# Autodesk Inventor assembly: GrampoParalelo
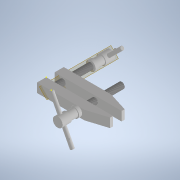
[picture p0: Inventor's stored thumbnail of the model, 180x180]
Saved by Autodesk Inventor 2021 (Build 250183000, 183)
## iProperties
Created: 2022-03-08
Part Number: GrampoParalelo
Document SubType Name: Assembly
Designer: aluno
Author: aluno
## Documents named in this file (6)
- E:\SENAI\Terceiro semestre\TPMC - Tecnololgia de produção mecatrônica\Grampo paralelo\GrampoParalelo.iam
- E:\SENAI\Terceiro semestre\TPMC - Tecnololgia de produção mecatrônica\Grampo paralelo\Garra2.ipt
- E:\SENAI\Terceiro semestre\TPMC - Tecnololgia de produção mecatrônica\Grampo paralelo\Parafuso2.ipt
- E:\SENAI\Terceiro semestre\TPMC - Tecnololgia de produção mecatrônica\Grampo paralelo\Garra1.ipt
- E:\SENAI\Terceiro semestre\TPMC - Tecnololgia de produção mecatrônica\Grampo paralelo\Parafuso1.ipt
- E:\SENAI\Terceiro semestre\TPMC - Tecnololgia de produção mecatrônica\Grampo paralelo\Manipulo.iam
## Components (6 placed, 5 different names)
1. Garra2:1 — Coincidente:1, Coincidente:3
2. Parafuso2:1 — Coincidente:1, Inserir:1, Tangente:1, Coincidente:6, Alinhado:2
3. Garra1:1 — Inserir:1, Coincidente:2, Coincidente:4, Tangente:1
4. Parafuso1:1 — Coincidente:2, Coincidente:3, Coincidente:4, Coincidente:5, Alinhado:1
5. Manipulo:1 [sub-assembly] — Coincidente:6, Alinhado:2
6. Manipulo:2 [sub-assembly] — Coincidente:5, Alinhado:1
## Relationships (10: Mate 6, Flush 2, Insert 1, Tangent 1)
- Coincidente:1 [Mate]: Garra2:1 ↔ Parafuso2:1
- Inserir:1: Parafuso2:1 ↔ Garra1:1
- Coincidente:2 [Mate]: Garra1:1 ↔ Parafuso1:1
- Coincidente:3 [Mate]: Garra2:1 ↔ Parafuso1:1
- Coincidente:4 [Mate]: Garra1:1 ↔ Parafuso1:1
- Tangente:1: Parafuso2:1 ↔ Garra1:1
- Coincidente:5 [Mate]: Parafuso1:1 ↔ Manipulo:2
- Alinhado:1 [Flush] (37.5 mm): Parafuso1:1 ↔ Manipulo:2
- Coincidente:6 [Mate]: Parafuso2:1 ↔ Manipulo:1
- Alinhado:2 [Flush] (37.5 mm): Parafuso2:1 ↔ Manipulo:1
